# Autodesk Inventor assembly: Wasp Omni Wheel Shaft
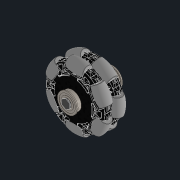
[picture p0: Inventor's stored thumbnail of the model, 180x180]
Saved by Autodesk Inventor 2022 (Build 260153000, 153)
## iProperties
Created: 2022-09-18
Part Number: Wasp Omni Wheel Shaft
Document SubType Name: Assembly
Designer: robpl
Author: robpl
## Documents named in this file (7)
- C:\Users\robpl\Downloads\22-20220924T142245Z-001\WASP 23-9-22\Workspaces\Workspace\Wasp Omni Wheel Shaft.iam
- C:\Users\robpl\Downloads\22-20220924T142245Z-001\WASP 23-9-22\Workspaces\Workspace\Wasp Omni Wheel Axle.ipt
- C:\Users\robpl\Downloads\22-20220924T142245Z-001\WASP 23-9-22\Workspaces\Workspace\0.5 Flanged Hex Bearing (1.125 OD) (217-3875).ipt
- C:\Users\robpl\Downloads\22-20220924T142245Z-001\WASP 23-9-22\Workspaces\Workspace\Omni Wheel\4_ Omni-Directional Wheel v2 (276-6194).iam
- C:\Users\robpl\Downloads\22-20220924T142245Z-001\WASP 23-9-22\Workspaces\Workspace\24T x 9mm Wide Double Flange Aluminum Pulley (HTD 5mm, 1_2” Hex Bore) (217-3227) (1).ipt
- C:\Users\robpl\Downloads\22-20220924T142245Z-001\WASP 23-9-22\Workspaces\Workspace\1mm 0.5in Hex Spacer.ipt
- C:\Users\robpl\Downloads\22-20220924T142245Z-001\WASP 23-9-22\Workspaces\Workspace\10mm E-Clip.ipt
## Components (10 placed, 6 different names)
1. Wasp Omni Wheel Axle:1 — Mate:1, Mate:2, Mate:3, Mate:4, Mate:6, Mate:7, Mate:8, Mate:9, Flush:2, Mate:20, Mate:21, Mate:22, Mate:23
2. 0.5 Flanged Hex Bearing (1.125 OD) (217-3875):1 — Mate:1, Mate:2, Flush:2, Mate:12, Mate:13, Mate:16
3. 0.5 Flanged Hex Bearing (1.125 OD) (217-3875):2 — Mate:3, Mate:4, Mate:19
4. 4_ Omni-Directional Wheel v2 (276-6194):1 [sub-assembly] — Mate:6, Mate:7, Mate:17, Mate:18
5. 24T x 9mm Wide Double Flange Aluminum Pulley (HTD 5mm, 1_2” Hex Bore) (217-3227) (1):1 — Mate:8, Mate:9, Mate:14, Mate:15
6. 1mm 0.5in Hex Spacer:1 — Mate:18, Mate:19
7. 1mm 0.5in Hex Spacer:2 — Mate:15, Mate:16, Mate:17
8. 1mm 0.5in Hex Spacer:3 — Mate:12, Mate:13, Mate:14
9. 10mm E-Clip:1 — Mate:20, Mate:21
10. 10mm E-Clip:2 — Mate:22, Mate:23
## Relationships (21: Mate 20, Flush 1)
- Mate:1: Wasp Omni Wheel Axle:1 ↔ 0.5 Flanged Hex Bearing (1.125 OD) (217-3875):1
- Mate:2: Wasp Omni Wheel Axle:1 ↔ 0.5 Flanged Hex Bearing (1.125 OD) (217-3875):1
- Mate:3: Wasp Omni Wheel Axle:1 ↔ 0.5 Flanged Hex Bearing (1.125 OD) (217-3875):2
- Mate:4: Wasp Omni Wheel Axle:1 ↔ 0.5 Flanged Hex Bearing (1.125 OD) (217-3875):2
- Mate:6: Wasp Omni Wheel Axle:1 ↔ 4_ Omni-Directional Wheel v2 (276-6194):1
- Mate:7: Wasp Omni Wheel Axle:1 ↔ 4_ Omni-Directional Wheel v2 (276-6194):1
- Mate:8: Wasp Omni Wheel Axle:1 ↔ 24T x 9mm Wide Double Flange Aluminum Pulley (HTD 5mm, 1_2” Hex Bore) (217-3227) (1):1
- Mate:9: Wasp Omni Wheel Axle:1 ↔ 24T x 9mm Wide Double Flange Aluminum Pulley (HTD 5mm, 1_2” Hex Bore) (217-3227) (1):1
- Flush:2: Wasp Omni Wheel Axle:1 ↔ 0.5 Flanged Hex Bearing (1.125 OD) (217-3875):1
- Mate:12: 0.5 Flanged Hex Bearing (1.125 OD) (217-3875):1 ↔ 1mm 0.5in Hex Spacer:3
- Mate:13: 0.5 Flanged Hex Bearing (1.125 OD) (217-3875):1 ↔ 1mm 0.5in Hex Spacer:3
- Mate:14: 24T x 9mm Wide Double Flange Aluminum Pulley (HTD 5mm, 1_2” Hex Bore) (217-3227) (1):1 ↔ 1mm 0.5in Hex Spacer:3
- Mate:15: 24T x 9mm Wide Double Flange Aluminum Pulley (HTD 5mm, 1_2” Hex Bore) (217-3227) (1):1 ↔ 1mm 0.5in Hex Spacer:2
- Mate:16: 0.5 Flanged Hex Bearing (1.125 OD) (217-3875):1 ↔ 1mm 0.5in Hex Spacer:2
- Mate:17: 4_ Omni-Directional Wheel v2 (276-6194):1 ↔ 1mm 0.5in Hex Spacer:2
- Mate:18: 4_ Omni-Directional Wheel v2 (276-6194):1 ↔ 1mm 0.5in Hex Spacer:1
- Mate:19: 0.5 Flanged Hex Bearing (1.125 OD) (217-3875):2 ↔ 1mm 0.5in Hex Spacer:1
- Mate:20: Wasp Omni Wheel Axle:1 ↔ 10mm E-Clip:1
- Mate:21: Wasp Omni Wheel Axle:1 ↔ 10mm E-Clip:1
- Mate:22: Wasp Omni Wheel Axle:1 ↔ 10mm E-Clip:2
- Mate:23: Wasp Omni Wheel Axle:1 ↔ 10mm E-Clip:2
